# Autodesk Inventor assembly: Caixa_10am_completa_v2
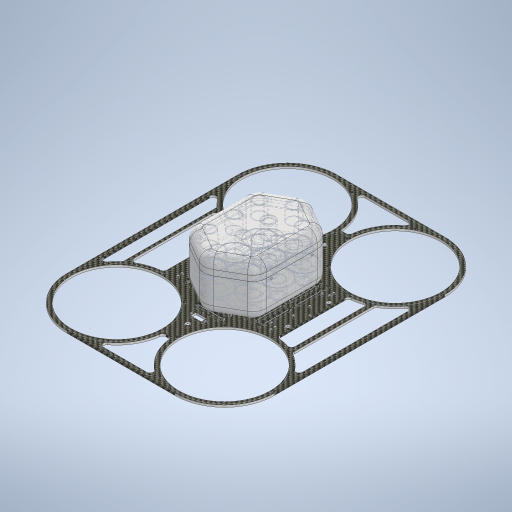
[picture p0: Inventor's stored thumbnail of the model, 512x512]
Saved by Autodesk Inventor 2024 (Build 280153000, 153)
## iProperties
Created: 2025-07-23
Part Number: Caixa_10am_completa_v2
Document SubType Name: Assembly
Designer: Bruno
Author: Bruno
## Documents named in this file (6)
- D:\Work\Research\Repositories\CybAer\DroneXixi\CAD_Caixa\Caixa_10am_completa_v2.iam
- D:\Work\Research\Repositories\CybAer\DroneXixi\CAD_Caixa\Caixa_10_amostras_v2.ipt
- D:\Work\Research\Repositories\CybAer\DroneXixi\CAD_Caixa\Separador_10_amostras_v2.ipt
- D:\Work\Research\Repositories\CybAer\DroneXixi\CAD_Caixa\Amostra_v1.ipt
- D:\Work\Research\Repositories\CybAer\DroneXixi\CAD_Caixa\Tampa_10_amostras_v2.ipt
- D:\Work\Research\Repositories\CybAer\DroneXixi\CAD\v3_top_carbon_fiber.ipt
## Components (5 placed, 5 different names)
1. Caixa_10_amostras_v2:1 — Mate:1, Mate:2, Tangent:1, Mate:3, Mate:4, Mate:5, Mate:7, Mate:8, Mate:9, Mate:10, Mate:11, Mate:12, Mate:13
2. Separador_10_amostras_v2:1 — Mate:3, Mate:4, Mate:5, Mate:6
3. Amostra_v1:1 — Mate:6, Mate:7
4. Tampa_10_amostras_v2:1 — Mate:8, Mate:9, Mate:10
5. v3_top_carbon_fiber:1 — Mate:11, Mate:12, Mate:13
## Relationships (14: Mate 13, Tangent 1)
- Mate:1: Caixa_10_amostras_v2:1
- Mate:2: Caixa_10_amostras_v2:1
- Tangent:1: Caixa_10_amostras_v2:1
- Mate:3: Caixa_10_amostras_v2:1 ↔ Separador_10_amostras_v2:1
- Mate:4: Caixa_10_amostras_v2:1 ↔ Separador_10_amostras_v2:1
- Mate:5: Caixa_10_amostras_v2:1 ↔ Separador_10_amostras_v2:1
- Mate:6 (0.1 mm): Separador_10_amostras_v2:1 ↔ Amostra_v1:1
- Mate:7: Caixa_10_amostras_v2:1 ↔ Amostra_v1:1
- Mate:8 (0.1 mm): Caixa_10_amostras_v2:1 ↔ Tampa_10_amostras_v2:1
- Mate:9: Caixa_10_amostras_v2:1 ↔ Tampa_10_amostras_v2:1
- Mate:10: Caixa_10_amostras_v2:1 ↔ Tampa_10_amostras_v2:1
- Mate:11: Caixa_10_amostras_v2:1 ↔ v3_top_carbon_fiber:1
- Mate:12: Caixa_10_amostras_v2:1 ↔ v3_top_carbon_fiber:1
- Mate:13: Caixa_10_amostras_v2:1 ↔ v3_top_carbon_fiber:1
